# Autodesk Inventor assembly: 전체형상
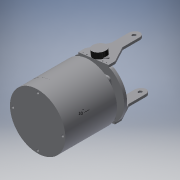
[picture p0: Inventor's stored thumbnail of the model, 180x180]
Saved by Autodesk Inventor 2018 (Build 220112000, 112)
## iProperties
Created: 2018-04-16
Part Number: 전체형상
Material: 일반
Document SubType Name: Assembly
Designer: CK
Author: CK
## Documents named in this file (3)
- C:\Users\CK\Desktop\캡스톤\전체형상.iam
- C:\Users\CK\Desktop\캡스톤\윗부분조립.iam
- C:\Users\CK\Desktop\캡스톤\바텀조립.iam
## Components (2 placed, 2 different names)
1. 윗부분조립:1 [sub-assembly] — 메이트:1, 메이트:2
2. 바텀조립:1 [sub-assembly] — 메이트:1, 메이트:2
## Relationships (2: Mate 2)
- 메이트:1 [Mate]: 윗부분조립:1 ↔ 바텀조립:1
- 메이트:2 [Mate]: 윗부분조립:1 ↔ 바텀조립:1
